# Autodesk Inventor assembly: 5
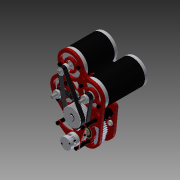
[picture p0: Inventor's stored thumbnail of the model, 180x180]
Saved by Autodesk Inventor 2013 (Build 170138000, 138)
## iProperties
Created: 2013-07-09
Part Number: 5
Document SubType Name: Assembly
Designer: mvarma
Author: mvarma
## Documents named in this file (54)
- C:\Users\mvarma\Desktop\GRT 2013-2014 Gearbox\Mark 5\Mark 5.iam
- C:\Users\mvarma\Desktop\GRT 2013-2014 Gearbox\Mark 5\Plates\Mounting Plate\Mounting Plate.ipt
- C:\Users\mvarma\Desktop\GRT 2013-2014 Gearbox\Mark 5\Plates\Cim Plate\Cim Plate.ipt
- C:\Users\mvarma\Desktop\GRT 2013-2014 Gearbox\Mark 5\Plates\Mounting Plate\Main Connecting Standoff Thick.ipt
- C:\Users\mvarma\Desktop\GRT 2013-2014 Gearbox\Mark 5\Plates\Mounting Plate\Main Connecting Standoff Thin.ipt
- C:\Users\mvarma\Desktop\GRT 2013-2014 Gearbox\Mark 5\Bearings\FR8-2RS.ipt
- C:\Users\mvarma\Desktop\GRT 2013-2014 Gearbox\Mark 5\Bearings\FR6-2RS.ipt
- C:\Users\mvarma\Desktop\GRT 2013-2014 Gearbox\Mark 5\Shafts\Cluster Shaft\15T 20DP - .375 Hex Bore.ipt
- C:\Users\mvarma\Desktop\GRT 2013-2014 Gearbox\Mark 5\Shafts\Cluster Shaft\28T 20DP - .375 Hex Bore.ipt
- C:\Users\mvarma\Desktop\GRT 2013-2014 Gearbox\Mark 5\Shafts\Cluster Shaft\Cluster Shaft Spacer.ipt
- C:\Users\mvarma\Desktop\GRT 2013-2014 Gearbox\Mark 5\Shafts\Cluster Shaft\Cluster Shaft.ipt
- C:\Users\mvarma\Desktop\GRT 2013-2014 Gearbox\Mark 5\Shafts\Cluster Shaft\Flexible Shaft Coupler 6208K411.ipt
- C:\Users\mvarma\Desktop\GRT 2013-2014 Gearbox\Mark 5\Encoder\Encoder Mount.ipt
- C:\Users\mvarma\Desktop\GRT 2013-2014 Gearbox\Mark 5\Encoder\S4-120-250-N-S-B.ipt
- C:\Users\mvarma\Desktop\GRT 2013-2014 Gearbox\Mark 5\Shafts\Output Shaft\Output Shaft Hex Sleave.ipt
- C:\Users\mvarma\Desktop\GRT 2013-2014 Gearbox\Mark 5\Shafts\Output Shaft\Output Shaft Insert.ipt
- C:\Users\mvarma\Desktop\GRT 2013-2014 Gearbox\Mark 5\Shafts\Output Shaft\Output Shaft.ipt
- C:\Users\mvarma\Desktop\GRT 2013-2014 Gearbox\Mark 5\Shafts\Output Shaft\35T 20DP - .188 Ball Shifting Bore.ipt
- C:\Users\mvarma\Desktop\GRT 2013-2014 Gearbox\Mark 5\Shafts\Output Shaft\48T 20DP - .188 Ball Shifting Bore.ipt
- C:\Users\mvarma\Desktop\GRT 2013-2014 Gearbox\Mark 5\Bearings\Thrust Bearing Washer - .6250 Bore.ipt
- C:\Users\mvarma\Desktop\GRT 2013-2014 Gearbox\Mark 5\Bearings\R10-Open.ipt
- C:\Users\mvarma\Desktop\GRT 2013-2014 Gearbox\Mark 5\Shafts\Output Shaft\Shim 10 thou .500 Bore.ipt
- C:\Users\mvarma\Desktop\GRT 2013-2014 Gearbox\Mark 5\Shafts\Output Shaft\Shim 10 thou .625 Bore.ipt
- C:\Users\mvarma\Desktop\GRT 2013-2014 Gearbox\Mark 5\Plates\Mounting Plate\10-32 Clinch Style Pem Nut .091 Minimum Panel Thickness.ipt
- C:\Users\mvarma\Desktop\GRT 2013-2014 Gearbox\Mark 5\Plates\Mounting Plate\.25-20 Clinch Style Pem Nut .125 Minimum Panel Thickness.ipt
- C:\Users\mvarma\Desktop\GRT 2013-2014 Gearbox\Mark 5\Motors\CIM Can.ipt
- C:\Users\mvarma\Desktop\GRT 2013-2014 Gearbox\Mark 5\Motors\Rotor.ipt
- C:\Users\mvarma\Desktop\GRT 2013-2014 Gearbox\Mark 5\Motors\Mini CIM Can.ipt
- C:\Users\mvarma\Desktop\GRT 2013-2014 Gearbox\Mark 5\Pulleys\16T 3mm GT2 - 8mm Key Broach.ipt
- C:\Users\mvarma\Desktop\GRT 2013-2014 Gearbox\Mark 5\Plates\Tensioning Shaft.ipt
- C:\Users\mvarma\Desktop\GRT 2013-2014 Gearbox\Mark 5\Bearings\R4-2RS.ipt
- C:\Users\mvarma\Desktop\GRT 2013-2014 Gearbox\Mark 5\Plates\Pneumatic Plate\Supporting Plate Standoff Long.ipt
- C:\Users\mvarma\Desktop\GRT 2013-2014 Gearbox\Mark 5\Plates\Pneumatic Plate\Supporting Plate Standoff Short.ipt
- C:\Users\mvarma\Desktop\GRT 2013-2014 Gearbox\Mark 5\Bolts\Socket Head Cap Screw 10-32 Thread 3.000 Length.ipt
- C:\Users\mvarma\Desktop\GRT 2013-2014 Gearbox\Mark 5\Bolts\Socket Head Cap Screw 10-32 Thread .750 Length.ipt
- C:\Users\mvarma\Desktop\GRT 2013-2014 Gearbox\Mark 5\Bolts\Socket Head Cap Screw 6-32 Thread 1.000 Length.ipt
- C:\Users\mvarma\Desktop\GRT 2013-2014 Gearbox\Mark 5\Pneumatic\Pancake Pneumatic.iam
- C:\Users\mvarma\Desktop\GRT 2013-2014 Gearbox\Mark 5\Pneumatic\Pneumatic Connector -Actuator Side.ipt
- C:\Users\mvarma\Desktop\GRT 2013-2014 Gearbox\Mark 5\Pneumatic\Pneumatic Connector -Shaft Side Cover.ipt
- C:\Users\mvarma\Desktop\GRT 2013-2014 Gearbox\Mark 5\Bolts\Socket Head Cap Screw 8-32 Thread .375 Length.ipt
- C:\Users\mvarma\Desktop\GRT 2013-2014 Gearbox\Mark 5\Bolts\Button Head Cap Screw 4-40 Thread .125 Length.ipt
- C:\Users\mvarma\Desktop\GRT 2013-2014 Gearbox\Mark 5\Bearings\R3-2RS.ipt
- C:\Users\mvarma\Desktop\GRT 2013-2014 Gearbox\Mark 5\Shafts\Ball Shifting Shaft.ipt
- C:\Users\mvarma\Desktop\GRT 2013-2014 Gearbox\Mark 5\.0625 Spring Pin .2500 Long.ipt
- C:\Users\mvarma\Desktop\GRT 2013-2014 Gearbox\Mark 5\Bolts\Socket Head Cap Screw 4-40 Thread 1.000 Length.ipt
- C:\Users\mvarma\Desktop\GRT 2013-2014 Gearbox\Mark 5\Plates\Pneumatic Plate\4-40 Clinch Style Pem Nut .091 Minimum Panel Thickness.ipt
- C:\Users\mvarma\Desktop\GRT 2013-2014 Gearbox\Mark 5\Bolts\Socket Head Cap Screw 10-32 Thread 1.500 Length.ipt
- C:\Users\mvarma\Desktop\GRT 2013-2014 Gearbox\Mark 5\Bolts\Socket Head Cap Screw 10-32 Thread 2.250 Length.ipt
- C:\Users\mvarma\Desktop\GRT 2013-2014 Gearbox\Mark 5\Plates\Pneumatic Plate\Pnuematic Plate.ipt
- C:\Users\mvarma\Desktop\GRT 2013-2014 Gearbox\Mark 5\Shafts\Cluster Shaft\Shim 10 thou .500 Bore.ipt
- C:\Users\mvarma\Desktop\GRT 2013-2014 Gearbox\Mark 5\Shafts\Cluster Shaft\48T 3mm GT2 - .500 Hex Broach - Hubless.ipt
- C:\Users\mvarma\Desktop\GRT 2013-2014 Gearbox\Mark 5\.500 spring clip.ipt
- C:\Users\mvarma\Desktop\GRT 2013-2014 Gearbox\Mark 5\Belts\267mm Belt.ipt
- C:\Users\mvarma\Desktop\GRT 2013-2014 Gearbox\Mark 5\Belts\285 mm Belt.ipt
## Components (79 placed, 52 different names)
1. Mounting Plate:1 — Mate:1, Mate:2, Mate:3, Mate:5, Mate:11, Mate:13, Mate:15, Mate:16, Mate:17, Mate:18, Mate:52, Mate:53, Mate:54, Mate:76, Mate:77, Mate:78, Mate:79, Mate:80, Mate:81, Mate:82, Mate:83, Mate:101, Mate:102
2. Cim Plate:1 — Mate:7, Mate:8, Mate:9, Mate:12, Mate:14, Mate:19, Mate:86, Mate:87, Mate:88, Mate:89, Mate:90, Mate:91, Mate:96, Mate:97, Mate:98, Mate:115, Mate:116, Mate:130, Mate:131, Mate:132, Mate:133, Mate:134, Mate:135, Mate:145, Mate:146, Mate:147, Mate:148, Mate:149, Mate:150, Mate:151, Mate:152, Mate:153, Mate:154, Mate:155, Mate:156, Mate:204
3. Main Connecting Standoff Thick:1 — Mate:5, Mate:8, Mate:18
4. Main Connecting Standoff Thick:2 — Mate:3, Mate:7, Mate:17, Mate:19
5. Main Connecting Standoff Thin:1 — Mate:1, Mate:2, Mate:9
6. FR8-2RS:1 — Mate:12, Mate:14, Mate:55, Mate:75
7. FR8-2RS:2 — Mate:11, Mate:13
8. FR6-2RS:1 — Mate:15, Mate:16, Mate:33, Mate:197
9. Cluster Shaft Spacer:1 — Mate:30, Mate:31, Mate:33, Mate:202
10. Cluster Shaft:1 — Mate:30, Mate:31, Mate:48, Mate:49, Mate:197, Mate:200, Mate:201, Mate:203, Mate:205, Mate:207, Mate:208, Mate:213, Mate:215, Mate:216, Mate:221
11. Flexible Shaft Coupler 6208K411:1 — Mate:48, Mate:49
12. Encoder Mount:1 — Mate:50, Mate:51, Mate:52, Mate:53, Mate:54, Mate:157, Mate:158, Mate:159, Mate:160
13. S4-120-250-N-S-B:1 — Mate:50, Mate:51
14. Output Shaft Hex Sleave:1 — Mate:58, Mate:59, Flush:1
15. Output Shaft Insert:1 — Mate:56, Mate:57
16. Output Shaft:1 — Mate:55, Mate:56, Mate:57, Mate:58, Mate:59, Flush:1, Mate:61, Mate:66, Mate:67, Mate:70, Flush:2, Mate:72, Mate:73, Mate:75
17. 35T 20DP - .188 Ball Shifting Bore:1 — Mate:60, Mate:61, Mate:64, Mate:65, Mate:68
18. 48T 20DP - .188 Ball Shifting Bore:1 — Mate:60, Mate:62, Mate:63, Mate:69
19. Thrust Bearing Washer - .6250 Bore:1 — Mate:67, Mate:69, Mate:71
20. Thrust Bearing Washer - .6250 Bore:2 — Mate:66, Mate:68, Mate:74
21. R10-Open:1 — Mate:62, Mate:63, Mate:74
22. R10-Open:2 — Mate:64, Mate:65
23. Shim 10 thou .500 Bore:1 — Mate:72, Mate:73
24. Shim 10 thou .625 Bore:1 — Mate:70, Mate:71, Flush:2
25. 10-32 Clinch Style Pem Nut .091 Minimum Panel Thickness:1 — Mate:77, Mate:80
26. 10-32 Clinch Style Pem Nut .091 Minimum Panel Thickness:2 — Mate:78, Mate:81
27. 10-32 Clinch Style Pem Nut .091 Minimum Panel Thickness:3 — Mate:76, Mate:79
28. .25-20 Clinch Style Pem Nut .125 Minimum Panel Thickness:1 — Mate:82, Mate:101
29. .25-20 Clinch Style Pem Nut .125 Minimum Panel Thickness:2 — Mate:83, Mate:102
30. CIM Can:1 — Mate:88, Mate:89, Mate:90, Mate:94, Mate:95
31. CIM Can:2 — Mate:86, Mate:87, Mate:91, Mate:92, Mate:93
32. Rotor:1 — Mate:94, Mate:95, Mate:105, Mate:225
33. Rotor:2 — Mate:92, Mate:93, Mate:103, Mate:226
34. Rotor:3 — Mate:99, Mate:100, Mate:107, Mate:222
35. Mini CIM Can:1 — Mate:96, Mate:97, Mate:98, Mate:99, Mate:100
36. 16T 3mm GT2 - 8mm Key Broach:1 — Mate:105, Mate:209
37. 16T 3mm GT2 - 8mm Key Broach:2 — Mate:107, Mate:211
38. 16T 3mm GT2 - 8mm Key Broach:3 — Mate:103, Mate:210
39. Tensioning Shaft:1 — Mate:115, Mate:116, Mate:119, Mate:120, Mate:186, Mate:187
40. R4-2RS:1 — Mate:117, Mate:118, Mate:119
41. R4-2RS:2 — Mate:117, Mate:118, Mate:120
42. Supporting Plate Standoff Long:1 — Mate:131, Mate:132
43. Supporting Plate Standoff Long:2 — Mate:130, Mate:133, Mate:189
44. Supporting Plate Standoff Short:1 — Mate:134, Mate:135, Mate:188, Mate:190
45. Socket Head Cap Screw 10-32 Thread 3.000 Length:1
46. Socket Head Cap Screw 10-32 Thread 3.000 Length:2
47. Socket Head Cap Screw 10-32 Thread .750 Length:1 — Mate:145, Mate:146
48. Socket Head Cap Screw 10-32 Thread .750 Length:2 — Mate:147, Mate:148
49. Socket Head Cap Screw 10-32 Thread .750 Length:3 — Mate:153, Mate:154
50. Socket Head Cap Screw 10-32 Thread .750 Length:4 — Mate:155, Mate:156
51. Socket Head Cap Screw 10-32 Thread .750 Length:5 — Mate:149, Mate:150
52. Socket Head Cap Screw 10-32 Thread .750 Length:6 — Mate:151, Mate:152
53. Socket Head Cap Screw 6-32 Thread 1.000 Length:1 — Mate:159, Mate:160
54. Socket Head Cap Screw 6-32 Thread 1.000 Length:2 — Mate:157, Mate:158
55. Pancake Pneumatic:1 [sub-assembly] — Mate:163, Mate:164, Mate:165, Mate:182, Mate:183, Mate:184, Mate:185, Mate:195, Mate:196
56. Pneumatic Connector -Actuator Side:1 — Mate:161, Mate:162, Mate:163, Mate:164, Mate:165, Mate:166, Mate:167, Flush:5, Mate:169, Mate:172, Mate:173
57. Pneumatic Connector -Shaft Side Cover:1 — Mate:166, Mate:167, Flush:5, Mate:168, Mate:170, Mate:171
58. Socket Head Cap Screw 8-32 Thread .375 Length:1 — Mate:161, Mate:162
59. Button Head Cap Screw 4-40 Thread .125 Length:1 — Mate:168, Mate:170
60. Button Head Cap Screw 4-40 Thread .125 Length:2 — Mate:169, Mate:171
61. R3-2RS:1 — Mate:172, Mate:173, Mate:174, Mate:177
62. Ball Shifting Shaft:1 — Mate:174, Mate:175, Mate:176, Mate:177
63. .0625 Spring Pin .2500 Long:1 — Mate:175, Mate:176
64. Socket Head Cap Screw 4-40 Thread 1.000 Length:1 — Mate:182, Mate:185
65. Socket Head Cap Screw 4-40 Thread 1.000 Length:2 — Mate:183, Mate:184
66. 4-40 Clinch Style Pem Nut .091 Minimum Panel Thickness:1 — Mate:192, Mate:193
67. 4-40 Clinch Style Pem Nut .091 Minimum Panel Thickness:2 — Mate:191, Mate:194
68. Socket Head Cap Screw 10-32 Thread 1.500 Length:1
69. Socket Head Cap Screw 10-32 Thread 2.250 Length:1 — Mate:186, Mate:187, Mate:224
70. Pnuematic Plate:1 — Mate:188, Mate:189, Mate:190, Mate:191, Mate:192, Mate:193, Mate:194, Mate:195, Mate:196
71. 15T 20DP - .375 Hex Bore:1 — Mate:198, Mate:199, Flush:8, Mate:200
72. 28T 20DP - .375 Hex Bore:1 — Mate:198, Mate:199, Flush:8, Mate:201, Mate:202
73. FR8-2RS:3 — Mate:203, Mate:204, Mate:206
74. Shim 10 thou .500 Bore:2 — Mate:205, Mate:206, Mate:214
75. 48T 3mm GT2 - .500 Hex Broach - Hubless:1 — Mate:208, Mate:211, Mate:212, Flush:9, Mate:213, Mate:223
76. 48T 3mm GT2 - .500 Hex Broach - Hubless:2 — Mate:207, Mate:209, Mate:210, Mate:212, Flush:9, Mate:214, Mate:220
77. .500 spring clip:1 — Mate:215, Mate:216
78. 267mm Belt:1 — Mate:220, Mate:224, Mate:225, Mate:226
79. 285 mm Belt:1 — Mate:221, Mate:222, Mate:223
## Relationships (167: Mate 162, Flush 5)
- Mate:1: Mounting Plate:1 ↔ Main Connecting Standoff Thin:1
- Mate:2: Mounting Plate:1 ↔ Main Connecting Standoff Thin:1
- Mate:3: Mounting Plate:1 ↔ Main Connecting Standoff Thick:2
- Mate:5: Mounting Plate:1 ↔ Main Connecting Standoff Thick:1
- Mate:7: Cim Plate:1 ↔ Main Connecting Standoff Thick:2
- Mate:8: Cim Plate:1 ↔ Main Connecting Standoff Thick:1
- Mate:9: Cim Plate:1 ↔ Main Connecting Standoff Thin:1
- Mate:11: Mounting Plate:1 ↔ FR8-2RS:2
- Mate:12: Cim Plate:1 ↔ FR8-2RS:1
- Mate:13: Mounting Plate:1 ↔ FR8-2RS:2
- Mate:14: Cim Plate:1 ↔ FR8-2RS:1
- Mate:15: Mounting Plate:1 ↔ FR6-2RS:1
- Mate:16: Mounting Plate:1 ↔ FR6-2RS:1
- Mate:17: Mounting Plate:1 ↔ Main Connecting Standoff Thick:2
- Mate:18: Mounting Plate:1 ↔ Main Connecting Standoff Thick:1
- Mate:19: Cim Plate:1 ↔ Main Connecting Standoff Thick:2
- Mate:30: Cluster Shaft Spacer:1 ↔ Cluster Shaft:1
- Mate:31: Cluster Shaft Spacer:1 ↔ Cluster Shaft:1
- Mate:33: FR6-2RS:1 ↔ Cluster Shaft Spacer:1
- Mate:48: Cluster Shaft:1 ↔ Flexible Shaft Coupler 6208K411:1
- Mate:49: Cluster Shaft:1 ↔ Flexible Shaft Coupler 6208K411:1
- Mate:50: Encoder Mount:1 ↔ S4-120-250-N-S-B:1
- Mate:51: Encoder Mount:1 ↔ S4-120-250-N-S-B:1
- Mate:52: Mounting Plate:1 ↔ Encoder Mount:1
- Mate:53: Mounting Plate:1 ↔ Encoder Mount:1
- Mate:54: Mounting Plate:1 ↔ Encoder Mount:1
- Mate:55: FR8-2RS:1 ↔ Output Shaft:1
- Mate:56: Output Shaft Insert:1 ↔ Output Shaft:1
- Mate:57: Output Shaft Insert:1 ↔ Output Shaft:1
- Mate:58: Output Shaft Hex Sleave:1 ↔ Output Shaft:1
- Mate:59: Output Shaft Hex Sleave:1 ↔ Output Shaft:1
- Flush:1: Output Shaft Hex Sleave:1 ↔ Output Shaft:1
- Mate:60: 35T 20DP - .188 Ball Shifting Bore:1 ↔ 48T 20DP - .188 Ball Shifting Bore:1
- Mate:61: Output Shaft:1 ↔ 35T 20DP - .188 Ball Shifting Bore:1
- Mate:62: 48T 20DP - .188 Ball Shifting Bore:1 ↔ R10-Open:1
- Mate:63: 48T 20DP - .188 Ball Shifting Bore:1 ↔ R10-Open:1
- Mate:64: 35T 20DP - .188 Ball Shifting Bore:1 ↔ R10-Open:2
- Mate:65: 35T 20DP - .188 Ball Shifting Bore:1 ↔ R10-Open:2
- Mate:66: Output Shaft:1 ↔ Thrust Bearing Washer - .6250 Bore:2
- Mate:67: Output Shaft:1 ↔ Thrust Bearing Washer - .6250 Bore:1
- Mate:68: 35T 20DP - .188 Ball Shifting Bore:1 ↔ Thrust Bearing Washer - .6250 Bore:2
- Mate:69: 48T 20DP - .188 Ball Shifting Bore:1 ↔ Thrust Bearing Washer - .6250 Bore:1
- Mate:70: Output Shaft:1 ↔ Shim 10 thou .625 Bore:1
- Mate:71: Thrust Bearing Washer - .6250 Bore:1 ↔ Shim 10 thou .625 Bore:1
- Flush:2: Output Shaft:1 ↔ Shim 10 thou .625 Bore:1
- Mate:72: Output Shaft:1 ↔ Shim 10 thou .500 Bore:1
- Mate:73: Output Shaft:1 ↔ Shim 10 thou .500 Bore:1
- Mate:74: Thrust Bearing Washer - .6250 Bore:2 ↔ R10-Open:1
- Mate:75: FR8-2RS:1 ↔ Output Shaft:1
- Mate:76: Mounting Plate:1 ↔ 10-32 Clinch Style Pem Nut .091 Minimum Panel Thickness:3
- Mate:77: Mounting Plate:1 ↔ 10-32 Clinch Style Pem Nut .091 Minimum Panel Thickness:1
- Mate:78: Mounting Plate:1 ↔ 10-32 Clinch Style Pem Nut .091 Minimum Panel Thickness:2
- Mate:79: Mounting Plate:1 ↔ 10-32 Clinch Style Pem Nut .091 Minimum Panel Thickness:3
- Mate:80: Mounting Plate:1 ↔ 10-32 Clinch Style Pem Nut .091 Minimum Panel Thickness:1
- Mate:81: Mounting Plate:1 ↔ 10-32 Clinch Style Pem Nut .091 Minimum Panel Thickness:2
- Mate:82: Mounting Plate:1 ↔ .25-20 Clinch Style Pem Nut .125 Minimum Panel Thickness:1
- Mate:83: Mounting Plate:1 ↔ .25-20 Clinch Style Pem Nut .125 Minimum Panel Thickness:2
- Mate:86: Cim Plate:1 ↔ CIM Can:2
- Mate:87: Cim Plate:1 ↔ CIM Can:2
- Mate:88: Cim Plate:1 ↔ CIM Can:1
- Mate:89: Cim Plate:1 ↔ CIM Can:1
- Mate:90: Cim Plate:1 ↔ CIM Can:1
- Mate:91: Cim Plate:1 ↔ CIM Can:2
- Mate:92: CIM Can:2 ↔ Rotor:2
- Mate:93: CIM Can:2 ↔ Rotor:2
- Mate:94: CIM Can:1 ↔ Rotor:1
- Mate:95: CIM Can:1 ↔ Rotor:1
- Mate:96: Cim Plate:1 ↔ Mini CIM Can:1
- Mate:97: Cim Plate:1 ↔ Mini CIM Can:1
- Mate:98: Cim Plate:1 ↔ Mini CIM Can:1
- Mate:99: Rotor:3 ↔ Mini CIM Can:1
- Mate:100: Rotor:3 ↔ Mini CIM Can:1
- Mate:101: Mounting Plate:1 ↔ .25-20 Clinch Style Pem Nut .125 Minimum Panel Thickness:1
- Mate:102: Mounting Plate:1 ↔ .25-20 Clinch Style Pem Nut .125 Minimum Panel Thickness:2
- Mate:103: Rotor:2 ↔ 16T 3mm GT2 - 8mm Key Broach:3
- Mate:105: Rotor:1 ↔ 16T 3mm GT2 - 8mm Key Broach:1
- Mate:107: Rotor:3 ↔ 16T 3mm GT2 - 8mm Key Broach:2
- Mate:115: Cim Plate:1 ↔ Tensioning Shaft:1
- Mate:116: Cim Plate:1 ↔ Tensioning Shaft:1
- Mate:117: R4-2RS:1 ↔ R4-2RS:2
- Mate:118: R4-2RS:1 ↔ R4-2RS:2
- Mate:119: Tensioning Shaft:1 ↔ R4-2RS:1
- Mate:120: Tensioning Shaft:1 ↔ R4-2RS:2
- Mate:130: Cim Plate:1 ↔ Supporting Plate Standoff Long:2
- Mate:131: Cim Plate:1 ↔ Supporting Plate Standoff Long:1
- Mate:132: Cim Plate:1 ↔ Supporting Plate Standoff Long:1
- Mate:133: Cim Plate:1 ↔ Supporting Plate Standoff Long:2
- Mate:134: Cim Plate:1 ↔ Supporting Plate Standoff Short:1
- Mate:135: Cim Plate:1 ↔ Supporting Plate Standoff Short:1
- Mate:145: Cim Plate:1 ↔ Socket Head Cap Screw 10-32 Thread .750 Length:1
- Mate:146: Cim Plate:1 ↔ Socket Head Cap Screw 10-32 Thread .750 Length:1
- Mate:147: Cim Plate:1 ↔ Socket Head Cap Screw 10-32 Thread .750 Length:2
- Mate:148: Cim Plate:1 ↔ Socket Head Cap Screw 10-32 Thread .750 Length:2
- Mate:149: Cim Plate:1 ↔ Socket Head Cap Screw 10-32 Thread .750 Length:5
- Mate:150: Cim Plate:1 ↔ Socket Head Cap Screw 10-32 Thread .750 Length:5
- Mate:151: Cim Plate:1 ↔ Socket Head Cap Screw 10-32 Thread .750 Length:6
- Mate:152: Cim Plate:1 ↔ Socket Head Cap Screw 10-32 Thread .750 Length:6
- Mate:153: Cim Plate:1 ↔ Socket Head Cap Screw 10-32 Thread .750 Length:3
- Mate:154: Cim Plate:1 ↔ Socket Head Cap Screw 10-32 Thread .750 Length:3
- Mate:155: Cim Plate:1 ↔ Socket Head Cap Screw 10-32 Thread .750 Length:4
- Mate:156: Cim Plate:1 ↔ Socket Head Cap Screw 10-32 Thread .750 Length:4
- Mate:157: Encoder Mount:1 ↔ Socket Head Cap Screw 6-32 Thread 1.000 Length:2
- Mate:158: Encoder Mount:1 ↔ Socket Head Cap Screw 6-32 Thread 1.000 Length:2
- Mate:159: Encoder Mount:1 ↔ Socket Head Cap Screw 6-32 Thread 1.000 Length:1
- Mate:160: Encoder Mount:1 ↔ Socket Head Cap Screw 6-32 Thread 1.000 Length:1
- Mate:161: Pneumatic Connector -Actuator Side:1 ↔ Socket Head Cap Screw 8-32 Thread .375 Length:1
- Mate:162: Pneumatic Connector -Actuator Side:1 ↔ Socket Head Cap Screw 8-32 Thread .375 Length:1
- Mate:163: Pancake Pneumatic:1 ↔ Pneumatic Connector -Actuator Side:1
- Mate:164: Pancake Pneumatic:1 ↔ Pneumatic Connector -Actuator Side:1
- Mate:165: Pancake Pneumatic:1 ↔ Pneumatic Connector -Actuator Side:1
- Mate:166: Pneumatic Connector -Actuator Side:1 ↔ Pneumatic Connector -Shaft Side Cover:1
- Mate:167: Pneumatic Connector -Actuator Side:1 ↔ Pneumatic Connector -Shaft Side Cover:1
- Flush:5: Pneumatic Connector -Actuator Side:1 ↔ Pneumatic Connector -Shaft Side Cover:1
- Mate:168: Pneumatic Connector -Shaft Side Cover:1 ↔ Button Head Cap Screw 4-40 Thread .125 Length:1
- Mate:169: Pneumatic Connector -Actuator Side:1 ↔ Button Head Cap Screw 4-40 Thread .125 Length:2
- Mate:170: Pneumatic Connector -Shaft Side Cover:1 ↔ Button Head Cap Screw 4-40 Thread .125 Length:1
- Mate:171: Pneumatic Connector -Shaft Side Cover:1 ↔ Button Head Cap Screw 4-40 Thread .125 Length:2
- Mate:172: Pneumatic Connector -Actuator Side:1 ↔ R3-2RS:1
- Mate:173: Pneumatic Connector -Actuator Side:1 ↔ R3-2RS:1
- Mate:174: R3-2RS:1 ↔ Ball Shifting Shaft:1
- Mate:175: Ball Shifting Shaft:1 ↔ .0625 Spring Pin .2500 Long:1
- Mate:176: Ball Shifting Shaft:1 ↔ .0625 Spring Pin .2500 Long:1
- Mate:177: R3-2RS:1 ↔ Ball Shifting Shaft:1
- Mate:182: Pancake Pneumatic:1 ↔ Socket Head Cap Screw 4-40 Thread 1.000 Length:1
- Mate:183: Pancake Pneumatic:1 ↔ Socket Head Cap Screw 4-40 Thread 1.000 Length:2
- Mate:184: Pancake Pneumatic:1 ↔ Socket Head Cap Screw 4-40 Thread 1.000 Length:2
- Mate:185: Pancake Pneumatic:1 ↔ Socket Head Cap Screw 4-40 Thread 1.000 Length:1
- Mate:186: Tensioning Shaft:1 ↔ Socket Head Cap Screw 10-32 Thread 2.250 Length:1
- Mate:187: Tensioning Shaft:1 ↔ Socket Head Cap Screw 10-32 Thread 2.250 Length:1
- Mate:188: Supporting Plate Standoff Short:1 ↔ Pnuematic Plate:1
- Mate:189: Supporting Plate Standoff Long:2 ↔ Pnuematic Plate:1
- Mate:190: Supporting Plate Standoff Short:1 ↔ Pnuematic Plate:1
- Mate:191: 4-40 Clinch Style Pem Nut .091 Minimum Panel Thickness:2 ↔ Pnuematic Plate:1
- Mate:192: 4-40 Clinch Style Pem Nut .091 Minimum Panel Thickness:1 ↔ Pnuematic Plate:1
- Mate:193: 4-40 Clinch Style Pem Nut .091 Minimum Panel Thickness:1 ↔ Pnuematic Plate:1
- Mate:194: 4-40 Clinch Style Pem Nut .091 Minimum Panel Thickness:2 ↔ Pnuematic Plate:1
- Mate:195: Pancake Pneumatic:1 ↔ Pnuematic Plate:1
- Mate:196: Pancake Pneumatic:1 ↔ Pnuematic Plate:1
- Mate:197: FR6-2RS:1 ↔ Cluster Shaft:1
- Mate:198: 15T 20DP - .375 Hex Bore:1 ↔ 28T 20DP - .375 Hex Bore:1
- Mate:199: 15T 20DP - .375 Hex Bore:1 ↔ 28T 20DP - .375 Hex Bore:1
- Flush:8: 15T 20DP - .375 Hex Bore:1 ↔ 28T 20DP - .375 Hex Bore:1
- Mate:200: Cluster Shaft:1 ↔ 15T 20DP - .375 Hex Bore:1
- Mate:201: Cluster Shaft:1 ↔ 28T 20DP - .375 Hex Bore:1
- Mate:202: Cluster Shaft Spacer:1 ↔ 28T 20DP - .375 Hex Bore:1
- Mate:203: Cluster Shaft:1 ↔ FR8-2RS:3
- Mate:204: Cim Plate:1 ↔ FR8-2RS:3
- Mate:205: Cluster Shaft:1 ↔ Shim 10 thou .500 Bore:2
- Mate:206: FR8-2RS:3 ↔ Shim 10 thou .500 Bore:2
- Mate:207: Cluster Shaft:1 ↔ 48T 3mm GT2 - .500 Hex Broach - Hubless:2
- Mate:208: Cluster Shaft:1 ↔ 48T 3mm GT2 - .500 Hex Broach - Hubless:1
- Mate:209: 16T 3mm GT2 - 8mm Key Broach:1 ↔ 48T 3mm GT2 - .500 Hex Broach - Hubless:2
- Mate:210: 16T 3mm GT2 - 8mm Key Broach:3 ↔ 48T 3mm GT2 - .500 Hex Broach - Hubless:2
- Mate:211: 16T 3mm GT2 - 8mm Key Broach:2 ↔ 48T 3mm GT2 - .500 Hex Broach - Hubless:1
- Mate:212: 48T 3mm GT2 - .500 Hex Broach - Hubless:1 ↔ 48T 3mm GT2 - .500 Hex Broach - Hubless:2
- Flush:9: 48T 3mm GT2 - .500 Hex Broach - Hubless:1 ↔ 48T 3mm GT2 - .500 Hex Broach - Hubless:2
- Mate:213: Cluster Shaft:1 ↔ 48T 3mm GT2 - .500 Hex Broach - Hubless:1
- Mate:214: Shim 10 thou .500 Bore:2 ↔ 48T 3mm GT2 - .500 Hex Broach - Hubless:2
- Mate:215: Cluster Shaft:1 ↔ .500 spring clip:1
- Mate:216 (0.0508 mm): Cluster Shaft:1 ↔ .500 spring clip:1
- Mate:220: 48T 3mm GT2 - .500 Hex Broach - Hubless:2 ↔ 267mm Belt:1
- Mate:221: Cluster Shaft:1 ↔ 285 mm Belt:1
- Mate:222: Rotor:3 ↔ 285 mm Belt:1
- Mate:223: 48T 3mm GT2 - .500 Hex Broach - Hubless:1 ↔ 285 mm Belt:1
- Mate:224: Socket Head Cap Screw 10-32 Thread 2.250 Length:1 ↔ 267mm Belt:1
- Mate:225: Rotor:1 ↔ 267mm Belt:1
- Mate:226: Rotor:2 ↔ 267mm Belt:1
